# Autodesk Inventor assembly: bay con 12
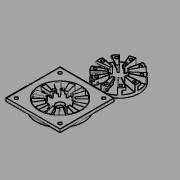
[picture p0: Inventor's stored thumbnail of the model, 180x180]
Saved by Autodesk Inventor 2015 (Build 190159000, 159)
## iProperties
Created: 2014-10-17
Part Number: bay con 12
Document SubType Name: Assembly
Designer: ericd_000
Author: ericd_000
## Documents named in this file (3)
- C:\Users\ericd_000\Dropbox\GitHub\initial_cad\eric_cad\bay con 12.iam
- C:\Users\ericd_000\Dropbox\GitHub\initial_cad\eric_cad\bayonet container 12.ipt
- C:\Users\ericd_000\Dropbox\GitHub\initial_cad\eric_cad\male bayonet connector 12.ipt
## Components (2 placed, 2 different names)
1. bayonet container 12:1 — Mate:2
2. male bayonet connector 12:1 — Mate:1
## Relationships (2: Mate 2)
- Mate:1: male bayonet connector 12:1
- Mate:2: bayonet container 12:1
